# Autodesk Inventor assembly: 01001 ASY GBK wall shield Center 10
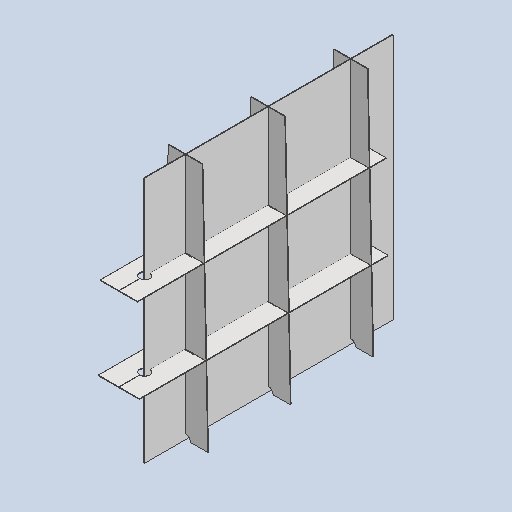
[picture p0: Inventor's stored thumbnail of the model, 512x512]
Saved by Autodesk Inventor 2026 (Build 300175000, 175)
## iProperties
Created: 2026-05-19
Part Number: 01001 ASY GBK wall shield Center 10
Document SubType Name: Assembly
Designer: pokla
Mass: 123029 g
Surface Area: 79995.2 cm^2
Volume: 15672.5 cm^3
Density: 7.85 g/cm^3
Author: admin
## Documents named in this file (5)
- C:\Users\pokla\Documents\Inventor\GBK-Gubkinskiy\01001 ASY GBK wall shield Center 10.iam
- C:\Users\pokla\Documents\Inventor\GBK-Gubkinskiy\01011 GBK Center rib 3.ipt
- C:\Users\pokla\Documents\Inventor\GBK-Gubkinskiy\01013 GBK stringer C7.ipt
- C:\Users\pokla\Documents\Inventor\GBK-Gubkinskiy\010.7 GBK shield.ipt
- C:\Users\pokla\Documents\Inventor\GBK-Gubkinskiy\01014 GBK stringer C8.ipt
## Components (11 placed, 4 different names)
1. 01013 GBK stringer C7.ipt:1 — Жесткий:1
2. 010.7 GBK shield.ipt:1 — Совмещение:1, Заподлицо:1, Совмещение:2, Совмещение:5, Заподлицо:5, Совмещение:4, Заподлицо:6, Заподлицо:7
3. 01014 GBK stringer C8.ipt:1 — Жесткий:2
4. 01013 GBK stringer C7.ipt:2 — Жесткий:4
5. 01014 GBK stringer C8.ipt:2 — Жесткий:3
6. 01011 GBK Center rib 3.ipt:1 — Совмещение:4, Заподлицо:4, Заподлицо:6, Жесткий:3, Жесткий:4
7. 01011 GBK Center rib 3.ipt:2 — Совмещение:5, Заподлицо:5, Заподлицо:4, Заподлицо:7, Жесткий:1, Жесткий:2
8. 01011 GBK Center rib 3.ipt:3
9. 01011 GBK Center rib 3.ipt:4
10. 01011 GBK Center rib 3.ipt:5
11. 01011 GBK Center rib 3.ipt:6
## Component patterns: (3 elements, first: 01011 GBK Center rib 3.ipt:1 + 01011 GBK Center rib 3.ipt:2)
## Relationships (13: Flush 5, Mate 4, WeldJoint 4)
- Совмещение:1 [Mate]: 010.7 GBK shield.ipt:1
- Заподлицо:1 [Flush]: 010.7 GBK shield.ipt:1
- Совмещение:2 [Mate]: 010.7 GBK shield.ipt:1
- Совмещение:5 [Mate]: 010.7 GBK shield.ipt:1 ↔ 01011 GBK Center rib 3.ipt:2
- Заподлицо:5 [Flush] (250 mm): 010.7 GBK shield.ipt:1 ↔ 01011 GBK Center rib 3.ipt:2
- Совмещение:4 [Mate]: 010.7 GBK shield.ipt:1 ↔ 01011 GBK Center rib 3.ipt:1
- Заподлицо:4 [Flush]: 01011 GBK Center rib 3.ipt:1 ↔ 01011 GBK Center rib 3.ipt:2
- Заподлицо:6 [Flush]: 010.7 GBK shield.ipt:1 ↔ 01011 GBK Center rib 3.ipt:1
- Заподлицо:7 [Flush]: 010.7 GBK shield.ipt:1 ↔ 01011 GBK Center rib 3.ipt:2
- Жесткий:1 [WeldJoint] (4 mm): 01013 GBK stringer C7.ipt:1 ↔ 01011 GBK Center rib 3.ipt:2
- Жесткий:2 [WeldJoint] (4 mm): 01014 GBK stringer C8.ipt:1 ↔ 01011 GBK Center rib 3.ipt:2
- Жесткий:3 [WeldJoint]: 01014 GBK stringer C8.ipt:2 ↔ 01011 GBK Center rib 3.ipt:1
- Жесткий:4 [WeldJoint]: 01013 GBK stringer C7.ipt:2 ↔ 01011 GBK Center rib 3.ipt:1
